# Autodesk Inventor assembly: LucasCharles Assembly Final
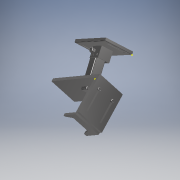
[picture p0: Inventor's stored thumbnail of the model, 180x180]
Saved by Autodesk Inventor 2018 (Build 220112000, 112)
## iProperties
Created: 2018-05-19
Part Number: LucasCharles Assembly Final
Document SubType Name: Assembly
Designer: Lucas
Author: Lucas
## Documents named in this file (10)
- C:\Users\Lucas\Documents\LucasCharles Assembly Final.iam
- C:\Users\Lucas\Documents\Part1.ipt
- C:\Users\Lucas\Documents\Part2.ipt
- C:\Users\Lucas\AppData\Local\Packages\Microsoft.MicrosoftEdge_8wekyb3d8bbwe\TempState\Downloads\LucasCharles Part 8 small nut.ipt
- C:\Users\Lucas\AppData\Local\Packages\Microsoft.MicrosoftEdge_8wekyb3d8bbwe\TempState\Downloads\LucasCharles Part 2 arm v2.ipt
- C:\Users\Lucas\AppData\Local\Packages\Microsoft.MicrosoftEdge_8wekyb3d8bbwe\TempState\Downloads\LucasCharles Part6 bolt for arm to speaker holder..ipt
- C:\Users\Lucas\AppData\Local\Packages\Microsoft.MicrosoftEdge_8wekyb3d8bbwe\TempState\Downloads\LucasCharles part 5 nut.ipt
- C:\Users\Lucas\AppData\Local\Packages\Microsoft.MicrosoftEdge_8wekyb3d8bbwe\TempState\Downloads\LucasCharles Part 1 wall mount FINAL.ipt
- C:\Users\Lucas\AppData\Local\Packages\Microsoft.MicrosoftEdge_8wekyb3d8bbwe\TempState\Downloads\LucasCharles Part 4 bolt to hold arm to wall mount.ipt
- C:\Users\Lucas\AppData\Local\Packages\Microsoft.MicrosoftEdge_8wekyb3d8bbwe\TempState\Downloads\LucasCharles Part7 bolt for height.ipt
## Components (12 placed, 9 different names)
1. Part1:1 — Mate:1, Flush:1, Mate:2, Mate:4, Mate:8, Mate:9, Mate:10, Mate:11, Mate:12
2. Part2:1 — Mate:1, Flush:1, Mate:3, Mate:5
3. LucasCharles Part 8 small nut:1 — Mate:4, Mate:5
4. LucasCharles Part 8 small nut:2 — Mate:2, Mate:3
5. LucasCharles Part 2 arm v2:1 — Mate:8, Mate:9, Mate:14, Mate:15
6. LucasCharles Part6 bolt for arm to speaker holder.:1 — Mate:10, Mate:11, Mate:13
7. LucasCharles part 5 nut:1 — Mate:12, Mate:13
8. LucasCharles Part 4 bolt to hold arm to wall mount:1 — Mate:16, Mate:17, Mate:19
9. LucasCharles Part 1 wall mount FINAL:1 — Mate:14, Mate:15, Mate:16, Mate:17, Mate:18, Mate:20, Mate:21, Mate:22
10. LucasCharles part 5 nut:2 — Mate:18, Mate:19
11. LucasCharles Part7 bolt for height:1 — Mate:20, Mate:21, Mate:23
12. LucasCharles Part 8 small nut:3 — Mate:22, Mate:23
## Relationships (22: Mate 21, Flush 1)
- Mate:1: Part1:1 ↔ Part2:1
- Flush:1: Part1:1 ↔ Part2:1
- Mate:2: Part1:1 ↔ LucasCharles Part 8 small nut:2
- Mate:3: Part2:1 ↔ LucasCharles Part 8 small nut:2
- Mate:4: Part1:1 ↔ LucasCharles Part 8 small nut:1
- Mate:5: Part2:1 ↔ LucasCharles Part 8 small nut:1
- Mate:8: Part1:1 ↔ LucasCharles Part 2 arm v2:1
- Mate:9: Part1:1 ↔ LucasCharles Part 2 arm v2:1
- Mate:10: Part1:1 ↔ LucasCharles Part6 bolt for arm to speaker holder.:1
- Mate:11: Part1:1 ↔ LucasCharles Part6 bolt for arm to speaker holder.:1
- Mate:12: Part1:1 ↔ LucasCharles part 5 nut:1
- Mate:13: LucasCharles Part6 bolt for arm to speaker holder.:1 ↔ LucasCharles part 5 nut:1
- Mate:14: LucasCharles Part 2 arm v2:1 ↔ LucasCharles Part 1 wall mount FINAL:1
- Mate:15: LucasCharles Part 2 arm v2:1 ↔ LucasCharles Part 1 wall mount FINAL:1
- Mate:16: LucasCharles Part 4 bolt to hold arm to wall mount:1 ↔ LucasCharles Part 1 wall mount FINAL:1
- Mate:17: LucasCharles Part 4 bolt to hold arm to wall mount:1 ↔ LucasCharles Part 1 wall mount FINAL:1
- Mate:18: LucasCharles Part 1 wall mount FINAL:1 ↔ LucasCharles part 5 nut:2
- Mate:19: LucasCharles Part 4 bolt to hold arm to wall mount:1 ↔ LucasCharles part 5 nut:2
- Mate:20: LucasCharles Part 1 wall mount FINAL:1 ↔ LucasCharles Part7 bolt for height:1
- Mate:21: LucasCharles Part 1 wall mount FINAL:1 ↔ LucasCharles Part7 bolt for height:1
- Mate:22: LucasCharles Part 1 wall mount FINAL:1 ↔ LucasCharles Part 8 small nut:3
- Mate:23: LucasCharles Part7 bolt for height:1 ↔ LucasCharles Part 8 small nut:3
